# Autodesk Inventor assembly: Assembly
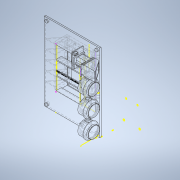
[picture p0: Inventor's stored thumbnail of the model, 180x180]
Saved by Autodesk Inventor 2020 (Build 240168000, 168)
## iProperties
Created: 2019-06-27
Part Number: Assembly
Document SubType Name: Assembly
Designer: jjsch
Author: jjsch
## Documents named in this file (8)
- C:\Users\jjsch\Documents\IIT\Coffee Project\coffee-is-a-core-value\hardware\Assembly.iam
- C:\Users\jjsch\Documents\IIT\Coffee Project\coffee-is-a-core-value\hardware\cam bien van tay.ipt
- C:\Users\jjsch\Documents\IIT\Coffee Project\coffee-is-a-core-value\hardware\lower casing.ipt
- C:\Users\jjsch\Documents\IIT\Coffee Project\coffee-is-a-core-value\hardware\upper casing.ipt
- C:\Users\jjsch\Documents\IIT\Coffee Project\coffee-is-a-core-value\hardware\Arcade Button_30mm.ipt
- C:\Users\jjsch\Documents\IIT\Coffee Project\coffee-is-a-core-value\hardware\top_casing.ipt
- C:\Users\jjsch\Documents\IIT\Coffee Project\coffee-is-a-core-value\hardware\rfid_top.ipt
- C:\Users\jjsch\Documents\IIT\Coffee Project\coffee-is-a-core-value\hardware\6D5L peg.ipt
## Components (12 placed, 7 different names)
1. cam bien van tay:1 — Mate:7, Mate:8, Mate:9
2. lower casing:1 — Mate:10, Flush:1, Flush:2
3. upper casing:1 — Mate:1, Mate:2, Mate:3, Mate:4, Mate:5, Mate:6, Mate:7, Mate:8, Mate:9, Mate:10, Flush:1, Flush:2, Mate:11, Flush:3, Flush:4
4. Arcade Button_30mm:1 — Mate:3, Mate:4
5. Arcade Button_30mm:2 — Mate:2, Mate:5
6. Arcade Button_30mm:3 — Mate:1, Mate:6
7. top_casing:1 — Mate:11, Flush:3, Flush:4, Mate:12, Flush:5, Flush:6, Mate:13, Flush:7, Mate:14, Mate:15, Mate:16, Flush:8, Flush:9, Flush:10
8. rfid_top:1 — Mate:12, Flush:5, Flush:6
9. 6D5L peg:1 — Mate:13, Flush:7
10. 6D5L peg:2 — Mate:14, Flush:9
11. 6D5L peg:3 — Mate:16, Flush:8
12. 6D5L peg:4 — Mate:15, Flush:10
## Relationships (26: Mate 16, Flush 10)
- Mate:1: upper casing:1 ↔ Arcade Button_30mm:3
- Mate:2: upper casing:1 ↔ Arcade Button_30mm:2
- Mate:3: upper casing:1 ↔ Arcade Button_30mm:1
- Mate:4: upper casing:1 ↔ Arcade Button_30mm:1
- Mate:5: upper casing:1 ↔ Arcade Button_30mm:2
- Mate:6: upper casing:1 ↔ Arcade Button_30mm:3
- Mate:7: cam bien van tay:1 ↔ upper casing:1
- Mate:8: cam bien van tay:1 ↔ upper casing:1
- Mate:9: cam bien van tay:1 ↔ upper casing:1
- Mate:10: lower casing:1 ↔ upper casing:1
- Flush:1: lower casing:1 ↔ upper casing:1
- Flush:2: lower casing:1 ↔ upper casing:1
- Mate:11: upper casing:1 ↔ top_casing:1
- Flush:3: upper casing:1 ↔ top_casing:1
- Flush:4: upper casing:1 ↔ top_casing:1
- Mate:12: top_casing:1 ↔ rfid_top:1
- Flush:5: top_casing:1 ↔ rfid_top:1
- Flush:6: top_casing:1 ↔ rfid_top:1
- Mate:13: top_casing:1 ↔ 6D5L peg:1
- Flush:7: top_casing:1 ↔ 6D5L peg:1
- Mate:14: top_casing:1 ↔ 6D5L peg:2
- Mate:15: top_casing:1 ↔ 6D5L peg:4
- Mate:16: top_casing:1 ↔ 6D5L peg:3
- Flush:8: top_casing:1 ↔ 6D5L peg:3
- Flush:9: top_casing:1 ↔ 6D5L peg:2
- Flush:10: top_casing:1 ↔ 6D5L peg:4
